# Autodesk Inventor assembly: Robotic arm attempt 2
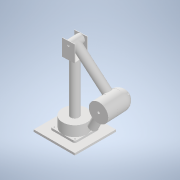
[picture p0: Inventor's stored thumbnail of the model, 180x180]
Saved by Autodesk Inventor 2020 (Build 240168000, 168)
## iProperties
Created: 2022-02-19
Part Number: Robotic arm attempt 2
Document SubType Name: Assembly
Designer: New-Computer
Author: New-Computer
## Documents named in this file (6)
- D:\Uni\FINAL YEAR\Semester 2\Robotics\Arm Design\2nd attempt\Robotic arm attempt 2.iam
- D:\Uni\FINAL YEAR\Semester 2\Robotics\Arm Design\2nd attempt\Base Plate 2.ipt
- D:\Uni\FINAL YEAR\Semester 2\Robotics\Arm Design\2nd attempt\Base Arm 2.ipt
- D:\Uni\FINAL YEAR\Semester 2\Robotics\Arm Design\2nd attempt\Intermediate Link 2.ipt
- D:\Uni\FINAL YEAR\Semester 2\Robotics\Arm Design\2nd attempt\End Link 2.ipt
- D:\Uni\FINAL YEAR\Semester 2\Robotics\Arm Design\2nd attempt\Wiring Cover 2.ipt
## Components (5 placed, 5 different names)
1. Base Plate 2:1 — Mate:3, Mate:7
2. Base Arm 2:1 — Mate:1, Mate:2, Mate:3, Mate:7
3. Intermediate Link 2:1 — Mate:1, Mate:2, Mate:5, Mate:6, Mate:8, Mate:9, Mate:10
4. End Link 2:1 — Mate:5, Mate:6
5. Wiring Cover 2:1 — Mate:8, Mate:9, Mate:10
## Relationships (9: Mate 9)
- Mate:1: Base Arm 2:1 ↔ Intermediate Link 2:1
- Mate:2 (0.5 mm): Base Arm 2:1 ↔ Intermediate Link 2:1
- Mate:3: Base Plate 2:1 ↔ Base Arm 2:1
- Mate:5: Intermediate Link 2:1 ↔ End Link 2:1
- Mate:6: Intermediate Link 2:1 ↔ End Link 2:1
- Mate:7: Base Plate 2:1 ↔ Base Arm 2:1
- Mate:8: Intermediate Link 2:1 ↔ Wiring Cover 2:1
- Mate:9: Intermediate Link 2:1 ↔ Wiring Cover 2:1
- Mate:10: Intermediate Link 2:1 ↔ Wiring Cover 2:1
